# Autodesk Inventor assembly: Riser Base
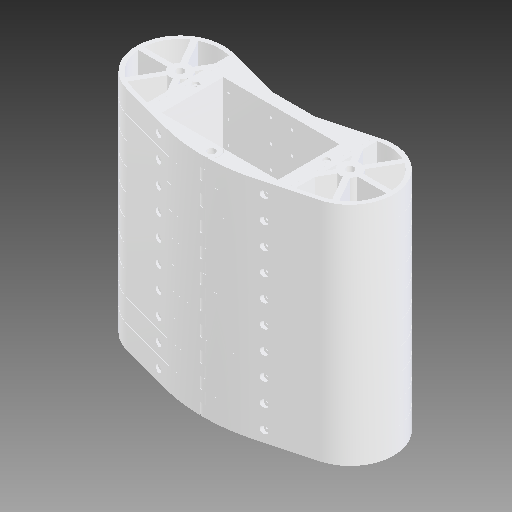
[picture p0: Inventor's stored thumbnail of the model, 512x512]
Saved by Autodesk Inventor 2017 SP1 (Build 210196100, 196)
## iProperties
Created: 2017-08-15
Part Number: Riser Base
Document SubType Name: Assembly
Designer: Zach
Author: Zach
## Documents named in this file (6)
- C:\Users\Zach\Documents\GitHub\tr1\src\Body\Chest Assembly\Rise Base Assembly\Riser Base.iam
- C:\Users\Zach\Documents\GitHub\tr1\src\Body\Chest Assembly\Rise Base Assembly\RB001.ipt
- C:\Users\Zach\Documents\GitHub\tr1\src\Body\Chest Assembly\Rise Base Assembly\RB002.ipt
- C:\Users\Zach\Documents\GitHub\tr1\src\Body\Chest Assembly\Rise Base Assembly\RB003.ipt
- C:\Users\Zach\Documents\GitHub\tr1\src\Body\Chest Assembly\Rise Base Assembly\RB004.ipt
- C:\Users\Zach\Documents\GitHub\tr1\src\Body\Chest Assembly\Rise Base Assembly\RB005.ipt
## Components (40 placed, 5 different names)
1. RB001:3 — Mate:73, Mate:102, Mate:103
2. RB002:3 — Mate:72
3. RB001:4
4. RB002:4 — Mate:71
5. RB001:5 — Mate:79, Mate:82
6. RB002:5 — Mate:78, Mate:81
7. RB001:6
8. RB002:6 — Mate:77, Mate:80
9. RB001:7 — Mate:85, Mate:88
10. RB002:7 — Mate:84, Mate:87
11. RB001:8
12. RB002:8 — Mate:83, Mate:86
13. RB001:9 — Mate:91
14. RB002:9 — Mate:90
15. RB001:10 — Mate:111, Mate:112, Mate:113
16. RB002:10 — Mate:89, Mate:114
17. RB001:11 — Mate:82, Mate:85
18. RB002:11 — Mate:81, Mate:84
19. RB001:12
20. RB002:12 — Mate:80, Mate:83
21. RB001:13 — Mate:88, Mate:91
22. RB002:13 — Mate:87, Mate:90
23. RB001:14
24. RB002:14 — Mate:86, Mate:89
25. RB001:15 — Mate:76, Mate:79
26. RB002:15 — Mate:75, Mate:78
27. RB001:16
28. RB002:16 — Mate:74, Mate:77
29. RB001:19 — Mate:73, Mate:76
30. RB002:19 — Mate:72, Mate:75
31. RB001:20
32. RB002:20 — Mate:71, Mate:74
33. RB003:1 — Mate:95, Mate:96, Mate:97, Mate:98, Mate:99, Mate:102, Mate:103
34. RB004:1 — Mate:100, Mate:101
35. RB005:1 — Mate:95, Mate:96, Mate:97
36. RB003:2 — Mate:98, Mate:99, Mate:100, Mate:101, Mate:115
37. RB003:3 — Flush:1, Flush:2, Mate:111, Mate:112, Mate:113
38. RB004:2 — Flush:3
39. RB005:2 — Flush:1, Mate:114
40. RB003:4 — Flush:2, Flush:3, Mate:116
## Relationships (94: Mate 91, Flush 3)
- [Mate]: RB001:3 ↔ RB001:4
- [Mate]: RB001:3 ↔ RB001:4
- [Mate]: RB001:4 ↔ RB002:4
- [Mate]: RB001:4 ↔ RB002:4
- [Mate]: RB001:3 ↔ RB002:3
- [Mate]: RB001:3 ↔ RB002:3
- [Mate]: RB001:5 ↔ RB001:6
- [Mate]: RB001:5 ↔ RB001:6
- [Mate]: RB001:6 ↔ RB002:6
- [Mate]: RB001:6 ↔ RB002:6
- [Mate]: RB001:5 ↔ RB002:5
- [Mate]: RB001:5 ↔ RB002:5
- [Mate]: RB001:7 ↔ RB001:8
- [Mate]: RB001:7 ↔ RB001:8
- [Mate]: RB001:8 ↔ RB002:8
- [Mate]: RB001:8 ↔ RB002:8
- [Mate]: RB001:7 ↔ RB002:7
- [Mate]: RB001:7 ↔ RB002:7
- [Mate]: RB001:9 ↔ RB001:10
- [Mate]: RB001:9 ↔ RB001:10
- [Mate]: RB001:10 ↔ RB002:10
- [Mate]: RB001:10 ↔ RB002:10
- [Mate]: RB001:9 ↔ RB002:9
- [Mate]: RB001:9 ↔ RB002:9
- [Mate]: RB001:11 ↔ RB001:12
- [Mate]: RB001:11 ↔ RB001:12
- [Mate]: RB001:12 ↔ RB002:12
- [Mate]: RB001:12 ↔ RB002:12
- [Mate]: RB001:11 ↔ RB002:11
- [Mate]: RB001:11 ↔ RB002:11
- [Mate]: RB001:13 ↔ RB001:14
- [Mate]: RB001:13 ↔ RB001:14
- [Mate]: RB001:14 ↔ RB002:14
- [Mate]: RB001:14 ↔ RB002:14
- [Mate]: RB001:13 ↔ RB002:13
- [Mate]: RB001:13 ↔ RB002:13
- [Mate]: RB001:15 ↔ RB001:16
- [Mate]: RB001:15 ↔ RB001:16
- [Mate]: RB001:16 ↔ RB002:16
- [Mate]: RB001:16 ↔ RB002:16
- [Mate]: RB001:15 ↔ RB002:15
- [Mate]: RB001:15 ↔ RB002:15
- [Mate]: RB001:19 ↔ RB001:20
- [Mate]: RB001:19 ↔ RB001:20
- [Mate]: RB001:20 ↔ RB002:20
- [Mate]: RB001:20 ↔ RB002:20
- [Mate]: RB001:19 ↔ RB002:19
- [Mate]: RB001:19 ↔ RB002:19
- Mate:71: RB002:4 ↔ RB002:20
- Mate:72: RB002:3 ↔ RB002:19
- Mate:73: RB001:3 ↔ RB001:19
- Mate:74: RB002:16 ↔ RB002:20
- Mate:75: RB002:15 ↔ RB002:19
- Mate:76: RB001:15 ↔ RB001:19
- Mate:77: RB002:6 ↔ RB002:16
- Mate:78: RB002:5 ↔ RB002:15
- Mate:79: RB001:5 ↔ RB001:15
- Mate:80: RB002:6 ↔ RB002:12
- Mate:81: RB002:5 ↔ RB002:11
- Mate:82: RB001:5 ↔ RB001:11
- Mate:83: RB002:8 ↔ RB002:12
- Mate:84: RB002:7 ↔ RB002:11
- Mate:85: RB001:7 ↔ RB001:11
- Mate:86: RB002:8 ↔ RB002:14
- Mate:87: RB002:7 ↔ RB002:13
- Mate:88: RB001:7 ↔ RB001:13
- Mate:89: RB002:10 ↔ RB002:14
- Mate:90: RB002:9 ↔ RB002:13
- Mate:91: RB001:9 ↔ RB001:13
- Mate:95: RB003:1 ↔ RB005:1
- Mate:96: RB003:1 ↔ RB005:1
- Mate:97: RB003:1 ↔ RB005:1
- Mate:98: RB003:1 ↔ RB003:2
- Mate:99: RB003:1 ↔ RB003:2
- Mate:100: RB004:1 ↔ RB003:2
- Mate:101: RB004:1 ↔ RB003:2
- Mate:102: RB001:3 ↔ RB003:1
- Mate:103: RB001:3 ↔ RB003:1
- [Mate]: RB003:3 ↔ RB005:2
- [Mate]: RB003:3 ↔ RB005:2
- [Mate]: RB003:3 ↔ RB005:2
- [Mate]: RB003:3 ↔ RB003:4
- [Mate]: RB003:3 ↔ RB003:4
- [Mate]: RB004:2 ↔ RB003:4
- [Mate]: RB004:2 ↔ RB003:4
- Flush:1: RB003:3 ↔ RB005:2
- Flush:2: RB003:3 ↔ RB003:4
- Flush:3: RB004:2 ↔ RB003:4
- Mate:111: RB001:10 ↔ RB003:3
- Mate:112: RB001:10 ↔ RB003:3
- Mate:113: RB001:10 ↔ RB003:3
- Mate:114: RB002:10 ↔ RB005:2
- Mate:115: RB003:2
- Mate:116: RB003:4
## Named parameters: d13_d4 = 0 mm, d14_d5 = 0 mm, d15_d6 = 0 mm, d16_d7 = 0 mm, d17_d8 = 0 mm, d18_d9 = 0 mm, d19_d13_d4 = 0 mm, d20_d14_d5 = 0 mm, d21_d15_d6 = 0 mm, d22_d16_d7 = 0 mm, d23_d17_d8 = 0 mm, d24_d18_d9 = 0 mm, d25_d13_d4 = 0 mm, d26_d14_d5 = 0 mm, d27_d15_d6 = 0 mm, d28_d16_d7 = 0 mm, d29_d17_d8 = 0 mm, d30_d18_d9 = 0 mm, d31_d13_d4 = 0 mm, d32_d14_d5 = 0 mm, d33_d15_d6 = 0 mm, d34_d16_d7 = 0 mm, d35_d17_d8 = 0 mm, d36_d18_d9 = 0 mm, d37_d13_d4 = 0 mm, d38_d14_d5 = 0 mm, d39_d15_d6 = 0 mm, d40_d16_d7 = 0 mm, d41_d17_d8 = 0 mm, d42_d18_d9 = 0 mm, d43_d13_d4 = 0 mm, d44_d14_d5 = 0 mm, d45_d15_d6 = 0 mm, d46_d16_d7 = 0 mm, d47_d17_d8 = 0 mm, d48_d18_d9 = 0 mm, d49_d13_d4 = 0 mm, d50_d14_d5 = 0 mm, d51_d15_d6 = 0 mm, d52_d16_d7 = 0 mm, d53_d17_d8 = 0 mm, d54_d18_d9 = 0 mm, d61_d13_d4 = 0 mm, d62_d14_d5 = 0 mm, d63_d15_d6 = 0 mm, d64_d16_d7 = 0 mm, d65_d17_d8 = 0 mm, d66_d18_d9 = 0 mm, d103_d95 = 0 mm, d104_d96 = 0 mm, d105_d97 = 0 mm, d106_d98 = 0 mm, d107_d99 = 0 mm, d108_d100 = 0 mm, d109_d94 = 0 mm
